# Autodesk Inventor assembly: CABEZAL
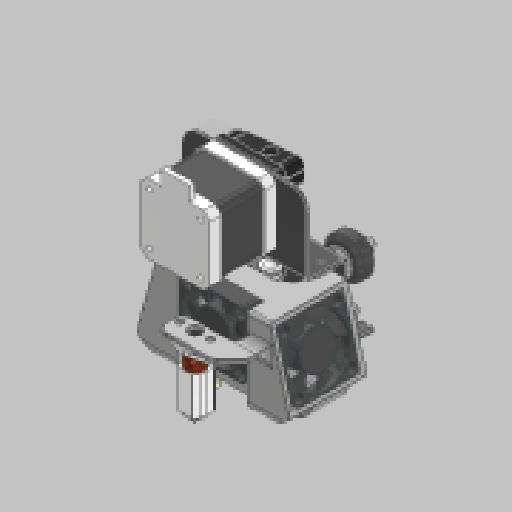
[picture p0: Inventor's stored thumbnail of the model, 512x512]
Saved by Autodesk Inventor 2025.3 (Build 293356000, 356)
## iProperties
Created: 2025-10-28
Part Number: CABEZAL
Document SubType Name: Assembly
Designer: Inema
Author: Inema
## Documents named in this file (6)
- C:\Users\Inema\OneDrive - INEMA S.A\Escritorio\Modelo Ender 3\CABEZAL.iam
- C:\Users\Inema\OneDrive - INEMA S.A\Escritorio\Modelo Ender 3\ASM Extruder.iam
- C:\Users\Inema\OneDrive - INEMA S.A\Escritorio\Modelo Ender 3\ASM Printing Head.iam
- C:\Users\Inema\OneDrive - INEMA S.A\Escritorio\Modelo Ender 3\mS_Ender_Dual_4010_1.1\mS_Ender_Dual_4010_1.1\mS_Ender_Dual_4010_1.1.ipt
- C:\Users\Inema\OneDrive - INEMA S.A\Escritorio\Modelo Ender 3\Nozzle fan.ipt
- C:\Users\Inema\OneDrive - INEMA S.A\Escritorio\Modelo Ender 3\3d-touch-v30.ipt
## Components (7 placed, 6 different names)
1. ASM Extruder_162 [sub-assembly]
2. ASM Printing Head_167 [sub-assembly]
3. mS_Ender_Dual_4010_1.1:1
4. Nozzle fan_172
5. Nozzle fan:2
6. Nozzle fan:3
7. 3d-touch-v30:1
## Relationships (14: Mate 12, Angle 1, Flush 1)
- [Mate]: ASM Extruder_162 ↔ ASM Printing Head_167
- [Angle] (180 deg): ASM Extruder_162 ↔ ASM Printing Head_167
- [Flush] (-1.45 mm): ASM Extruder_162 ↔ ASM Printing Head_167
- [Mate] (21 mm): ASM Printing Head_167 ↔ mS_Ender_Dual_4010_1.1:1
- [Mate]: mS_Ender_Dual_4010_1.1:1 ↔ Nozzle fan_172
- [Mate]: mS_Ender_Dual_4010_1.1:1 ↔ Nozzle fan_172
- [Mate]: mS_Ender_Dual_4010_1.1:1 ↔ Nozzle fan_172
- [Mate]: mS_Ender_Dual_4010_1.1:1 ↔ Nozzle fan:2
- [Mate] (0.5 mm): mS_Ender_Dual_4010_1.1:1 ↔ Nozzle fan:2
- [Mate] (0.5 mm): mS_Ender_Dual_4010_1.1:1 ↔ Nozzle fan:2
- [Mate] (0.5 mm): mS_Ender_Dual_4010_1.1:1 ↔ Nozzle fan:3
- [Mate] (0.5 mm): mS_Ender_Dual_4010_1.1:1 ↔ Nozzle fan:3
- [Mate]: mS_Ender_Dual_4010_1.1:1 ↔ Nozzle fan:3
- [Mate]: ASM Printing Head_167 ↔ mS_Ender_Dual_4010_1.1:1
## Named parameters: d31_d20 = 0 mm, d32_d21 = 0 mm, d33_d22 = 0.5 mm, d34_d23 = 0.5 mm, d36_d26 = 0.5 mm, d37_d27 = 0 mm
